# Autodesk Inventor assembly: dsitributor
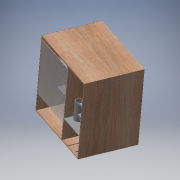
[picture p0: Inventor's stored thumbnail of the model, 180x180]
Saved by Autodesk Inventor 2019 (Build 230136000, 136)
## iProperties
Created: 2018-12-03
Part Number: dsitributor
Document SubType Name: Assembly
Designer: Bienvenue
Author: Bienvenue
## Documents named in this file (25)
- C:\Users\pouey\Desktop\rep3dM\distributeur.iam
- C:\Users\pouey\Desktop\rep3dM\planche_gauche.ipt
- C:\Users\pouey\Desktop\rep3dM\planche derrière.ipt
- C:\Users\pouey\Desktop\rep3dM\planche_bas.ipt
- C:\Users\pouey\Desktop\rep3dM\cloison_porte-monnayeur.ipt
- C:\Users\pouey\Desktop\rep3dM\monnayeur.ipt
- C:\Users\pouey\Desktop\rep3dM\cale_monnayeur.ipt
- C:\Users\pouey\Desktop\rep3dM\toboggan.ipt
- C:\Users\pouey\Desktop\rep3dM\tube.ipt
- C:\Users\pouey\Desktop\rep3dM\vis infini.ipt
- C:\Users\pouey\Desktop\rep3dM\piece-interieur-2.ipt
- C:\Users\pouey\Desktop\rep3dM\Pièce-interieur-3.ipt
- C:\Users\pouey\Desktop\rep3dM\Pièce-moteur-vis.ipt
- C:\Users\pouey\Desktop\rep3dM\vis infini_CPY.ipt
- C:\Users\pouey\Desktop\rep3dM\Pièce-moteur-vis_CPY.ipt
- C:\Users\pouey\Desktop\rep3dM\vis infini_CPY1.ipt
- C:\Users\pouey\Desktop\rep3dM\Pièce-moteur-vis_CPY1.ipt
- C:\Users\pouey\Desktop\rep3dM\vis infini_CPY2.ipt
- C:\Users\pouey\Desktop\rep3dM\Pièce-moteur-vis_CPY2.ipt
- C:\Users\pouey\Desktop\rep3dM\face-avant.ipt
- C:\Users\pouey\Desktop\rep3dM\piece-interieur4.ipt
- C:\Users\pouey\Desktop\rep3dM\vitre-avant.ipt
- C:\Users\pouey\Desktop\rep3dM\cale-moteur.ipt
- C:\Users\pouey\Desktop\rep3dM\tube-rend-monnaie.ipt
- C:\Users\pouey\Desktop\rep3dM\rampe-rendmonnaie.ipt
## Components (35 placed, 24 different names)
1. planche_gauche:1 — Mate:1, Flush:1, Flush:3, Flush:6, Mate:4, Mate:7, Placage:30, Placage:33, Placage:38, Placage:58, Placage:64, Placage:76, Placage:85
2. planche_gauche:2 — Mate:2, Flush:2, Flush:4, Flush:5, Flush:11, Placage:14, Placage:17, Placage:18, Placage:67, Placage:70, Tangente:7, Placage:90
3. planche derrière:1 — Mate:3, Flush:5, Flush:6, Mate:4, Flush:10, Placage:15, Placage:19, Placage:20, Placage:29, Placage:35, Placage:37, Placage:51, Placage:52, Placage:53, Placage:54, Placage:65, Placage:68, Placage:69, Placage:74, Placage:75, Placage:78, Placage:81, Placage:84, Tangente:6, Placage:88
4. planche_bas:1 — Mate:1, Mate:2, Flush:1, Flush:2, Flush:3, Flush:4, Mate:3, Angle:3, Placage:31, Placage:34, Placage:71, Placage:89
5. planche_bas:2 — Mate:7, Flush:10, Flush:11, Placage:16, Angle:2, Placage:21, Placage:22, Placage:57, Placage:63, Placage:77, Placage:80, Placage:87
6. cloison_porte-monnayeur:1 — Placage:14, Placage:15, Placage:16, Tangente:1, Tangente:2, Tangente:3, Tangente:4, Tangente:5, Placage:62
7. monnayeur:1 — Mate:11, Flush:14, Mate:13
8. cale_monnayeur:1 — Mate:11, Flush:14, Mate:13, Placage:17, Angle:2, Placage:19, Placage:21
9. toboggan:1 — Placage:18, Angle:3, Placage:20, Placage:22, Placage:24, Placage:25, Placage:26, Placage:27, Placage:28, Placage:66
10. tube:1 — Tangente:1, Placage:25
11. tube:2 — Placage:24, Tangente:2
12. tube:3 — Placage:26, Tangente:3
13. tube:4 — Placage:27, Tangente:4
14. tube:5 — Placage:28, Tangente:5
15. vis infini:1 — Placage:39, Placage:40, Placage:41, Angle:4, Angle:5
16. piece-interieur-2:1 — Placage:29, Placage:30, Placage:31, Placage:56, Placage:59, Placage:61, Placage:83, Placage:86
17. piece-interieur-2:2 — Placage:33, Placage:34, Placage:35, Placage:36
18. Pièce-interieur-3:1 — Placage:36, Placage:37, Placage:38, Placage:55, Placage:60, Placage:79, Placage:82
19. Pièce-moteur-vis:1 — Placage:39, Placage:40, Placage:41, Angle:4, Angle:5, Placage:51, Placage:59, Placage:60
20. vis infini_CPY:1 — Angle:6, Angle:7, Placage:42, Placage:43, Placage:44
21. Pièce-moteur-vis_CPY:1 — Angle:6, Angle:7, Placage:42, Placage:43, Placage:44, Placage:52, Placage:57, Placage:58
22. vis infini_CPY1:1 — Angle:8, Angle:9, Placage:45, Placage:46, Placage:47
23. Pièce-moteur-vis_CPY1:1 — Angle:8, Angle:9, Placage:45, Placage:46, Placage:47, Placage:53, Placage:55, Placage:56
24. vis infini_CPY2:1 — Angle:10, Angle:11, Placage:48, Placage:49, Placage:50
25. Pièce-moteur-vis_CPY2:1 — Angle:10, Angle:11, Placage:48, Placage:49, Placage:50, Placage:54, Placage:61, Placage:62
26. face-avant:1 — Placage:63, Placage:64, Placage:65, Placage:72, Placage:73
27. cale_monnayeur:2 — Placage:66, Placage:67, Placage:68
28. piece-interieur4:1 — Placage:69, Placage:70, Placage:71
29. vitre-avant:1 — Placage:72, Placage:73, Placage:74
30. cale-moteur:1 — Placage:75, Placage:76, Placage:77
31. cale-moteur:2 — Placage:78, Placage:79, Placage:80
32. cale-moteur:3 — Placage:84, Placage:85, Placage:86
33. cale-moteur:4 — Placage:81, Placage:82, Placage:83
34. tube-rend-monnaie:1 — Tangente:6, Tangente:7, Placage:87
35. rampe-rendmonnaie:1 — Placage:88, Placage:89, Placage:90
## Relationships (108: Mate 82, Angle 10, Flush 9, Tangent 7)
- Mate:1: planche_gauche:1 ↔ planche_bas:1
- Mate:2: planche_gauche:2 ↔ planche_bas:1
- Flush:1: planche_gauche:1 ↔ planche_bas:1
- Flush:2: planche_gauche:2 ↔ planche_bas:1
- Flush:3: planche_gauche:1 ↔ planche_bas:1
- Flush:4: planche_gauche:2 ↔ planche_bas:1
- Mate:3: planche derrière:1 ↔ planche_bas:1
- Flush:5: planche_gauche:2 ↔ planche derrière:1
- Flush:6: planche_gauche:1 ↔ planche derrière:1
- Mate:4: planche_gauche:1 ↔ planche derrière:1
- Mate:7: planche_gauche:1 ↔ planche_bas:2
- Flush:10: planche derrière:1 ↔ planche_bas:2
- Flush:11: planche_gauche:2 ↔ planche_bas:2
- Mate:11: monnayeur:1 ↔ cale_monnayeur:1
- Flush:14 (-50.8 mm): monnayeur:1 ↔ cale_monnayeur:1
- Mate:13: monnayeur:1 ↔ cale_monnayeur:1
- Placage:14 [Mate] (150 mm): planche_gauche:2 ↔ cloison_porte-monnayeur:1
- Placage:15 [Mate]: planche derrière:1 ↔ cloison_porte-monnayeur:1
- Placage:16 [Mate]: planche_bas:2 ↔ cloison_porte-monnayeur:1
- Placage:17 [Mate]: planche_gauche:2 ↔ cale_monnayeur:1
- Angle:2 (160 deg): planche_bas:2 ↔ cale_monnayeur:1
- Placage:18 [Mate]: planche_gauche:2 ↔ toboggan:1
- Angle:3 (180 deg): planche_bas:1 ↔ toboggan:1
- Placage:19 [Mate]: planche derrière:1 ↔ cale_monnayeur:1
- Placage:20 [Mate] (60 mm): planche derrière:1 ↔ toboggan:1
- Placage:21 [Mate] (50 mm): planche_bas:2 ↔ cale_monnayeur:1
- Placage:22 [Mate] (180 mm): planche_bas:2 ↔ toboggan:1
- Tangente:1 (10 mm): cloison_porte-monnayeur:1 ↔ tube:1
- Placage:24 [Mate]: toboggan:1 ↔ tube:2
- Tangente:2 (10 mm): cloison_porte-monnayeur:1 ↔ tube:2
- Placage:25 [Mate]: toboggan:1 ↔ tube:1
- Placage:26 [Mate]: toboggan:1 ↔ tube:3
- Tangente:3 (10 mm): cloison_porte-monnayeur:1 ↔ tube:3
- Placage:27 [Mate]: toboggan:1 ↔ tube:4
- Tangente:4 (10 mm): cloison_porte-monnayeur:1 ↔ tube:4
- Placage:28 [Mate]: toboggan:1 ↔ tube:5
- Tangente:5 (10 mm): cloison_porte-monnayeur:1 ↔ tube:5
- Placage:29 [Mate]: planche derrière:1 ↔ piece-interieur-2:1
- Placage:30 [Mate]: planche_gauche:1 ↔ piece-interieur-2:1
- Placage:31 [Mate] (250 mm): planche_bas:1 ↔ piece-interieur-2:1
- Placage:33 [Mate]: planche_gauche:1 ↔ piece-interieur-2:2
- Placage:34 [Mate] (100 mm): planche_bas:1 ↔ piece-interieur-2:2
- Placage:35 [Mate]: planche derrière:1 ↔ piece-interieur-2:2
- Placage:36 [Mate]: piece-interieur-2:2 ↔ Pièce-interieur-3:1
- Placage:37 [Mate]: planche derrière:1 ↔ Pièce-interieur-3:1
- Placage:38 [Mate] (125 mm): planche_gauche:1 ↔ Pièce-interieur-3:1
- Placage:39 [Mate]: vis infini:1 ↔ Pièce-moteur-vis:1
- Placage:40 [Mate] (-15 mm): vis infini:1 ↔ Pièce-moteur-vis:1
- Placage:41 [Mate] (5 mm): vis infini:1 ↔ Pièce-moteur-vis:1
- Angle:4 (0 deg): vis infini:1 ↔ Pièce-moteur-vis:1
- Angle:5 (90 deg): vis infini:1 ↔ Pièce-moteur-vis:1
- Angle:6 (90 deg): vis infini_CPY:1 ↔ Pièce-moteur-vis_CPY:1
- Angle:7 (0 deg): vis infini_CPY:1 ↔ Pièce-moteur-vis_CPY:1
- Placage:42 [Mate] (5 mm): vis infini_CPY:1 ↔ Pièce-moteur-vis_CPY:1
- Placage:43 [Mate] (-15 mm): vis infini_CPY:1 ↔ Pièce-moteur-vis_CPY:1
- Placage:44 [Mate]: vis infini_CPY:1 ↔ Pièce-moteur-vis_CPY:1
- Angle:8 (90 deg): vis infini_CPY1:1 ↔ Pièce-moteur-vis_CPY1:1
- Angle:9 (0 deg): vis infini_CPY1:1 ↔ Pièce-moteur-vis_CPY1:1
- Placage:45 [Mate] (5 mm): vis infini_CPY1:1 ↔ Pièce-moteur-vis_CPY1:1
- Placage:46 [Mate] (-15 mm): vis infini_CPY1:1 ↔ Pièce-moteur-vis_CPY1:1
- Placage:47 [Mate]: vis infini_CPY1:1 ↔ Pièce-moteur-vis_CPY1:1
- Angle:10 (90 deg): vis infini_CPY2:1 ↔ Pièce-moteur-vis_CPY2:1
- Angle:11 (0 deg): vis infini_CPY2:1 ↔ Pièce-moteur-vis_CPY2:1
- Placage:48 [Mate] (5 mm): vis infini_CPY2:1 ↔ Pièce-moteur-vis_CPY2:1
- Placage:49 [Mate] (-15 mm): vis infini_CPY2:1 ↔ Pièce-moteur-vis_CPY2:1
- Placage:50 [Mate]: vis infini_CPY2:1 ↔ Pièce-moteur-vis_CPY2:1
- Placage:51 [Mate] (40 mm): planche derrière:1 ↔ Pièce-moteur-vis:1
- Placage:52 [Mate] (40 mm): planche derrière:1 ↔ Pièce-moteur-vis_CPY:1
- Placage:53 [Mate] (40 mm): planche derrière:1 ↔ Pièce-moteur-vis_CPY1:1
- Placage:54 [Mate] (40 mm): planche derrière:1 ↔ Pièce-moteur-vis_CPY2:1
- Placage:55 [Mate] (20 mm): Pièce-interieur-3:1 ↔ Pièce-moteur-vis_CPY1:1
- Placage:56 [Mate] (30 mm): piece-interieur-2:1 ↔ Pièce-moteur-vis_CPY1:1
- Placage:57 [Mate] (40 mm): planche_bas:2 ↔ Pièce-moteur-vis_CPY:1
- Placage:58 [Mate] (25 mm): planche_gauche:1 ↔ Pièce-moteur-vis_CPY:1
- Placage:59 [Mate] (40 mm): piece-interieur-2:1 ↔ Pièce-moteur-vis:1
- Placage:60 [Mate] (25 mm): Pièce-interieur-3:1 ↔ Pièce-moteur-vis:1
- Placage:61 [Mate] (40 mm): piece-interieur-2:1 ↔ Pièce-moteur-vis_CPY2:1
- Placage:62 [Mate] (25 mm): cloison_porte-monnayeur:1 ↔ Pièce-moteur-vis_CPY2:1
- Placage:63 [Mate]: planche_bas:2 ↔ face-avant:1
- Placage:64 [Mate]: planche_gauche:1 ↔ face-avant:1
- Placage:65 [Mate] (300 mm): planche derrière:1 ↔ face-avant:1
- Placage:66 [Mate]: toboggan:1 ↔ cale_monnayeur:2
- Placage:67 [Mate]: planche_gauche:2 ↔ cale_monnayeur:2
- Placage:68 [Mate]: planche derrière:1 ↔ cale_monnayeur:2
- Placage:69 [Mate]: planche derrière:1 ↔ piece-interieur4:1
- Placage:70 [Mate]: planche_gauche:2 ↔ piece-interieur4:1
- Placage:71 [Mate] (115 mm): planche_bas:1 ↔ piece-interieur4:1
- Placage:72 [Mate]: face-avant:1 ↔ vitre-avant:1
- Placage:73 [Mate]: face-avant:1 ↔ vitre-avant:1
- Placage:74 [Mate] (300 mm): planche derrière:1 ↔ vitre-avant:1
- Placage:75 [Mate]: planche derrière:1 ↔ cale-moteur:1
- Placage:76 [Mate]: planche_gauche:1 ↔ cale-moteur:1
- Placage:77 [Mate]: planche_bas:2 ↔ cale-moteur:1
- Placage:78 [Mate]: planche derrière:1 ↔ cale-moteur:2
- Placage:79 [Mate]: Pièce-interieur-3:1 ↔ cale-moteur:2
- Placage:80 [Mate]: planche_bas:2 ↔ cale-moteur:2
- Placage:81 [Mate]: planche derrière:1 ↔ cale-moteur:4
- Placage:82 [Mate]: Pièce-interieur-3:1 ↔ cale-moteur:4
- Placage:83 [Mate]: piece-interieur-2:1 ↔ cale-moteur:4
- Placage:84 [Mate]: planche derrière:1 ↔ cale-moteur:3
- Placage:85 [Mate]: planche_gauche:1 ↔ cale-moteur:3
- Placage:86 [Mate]: piece-interieur-2:1 ↔ cale-moteur:3
- Tangente:6: planche derrière:1 ↔ tube-rend-monnaie:1
- Tangente:7: planche_gauche:2 ↔ tube-rend-monnaie:1
- Placage:87 [Mate] (170 mm): planche_bas:2 ↔ tube-rend-monnaie:1
- Placage:88 [Mate]: planche derrière:1 ↔ rampe-rendmonnaie:1
- Placage:89 [Mate]: planche_bas:1 ↔ rampe-rendmonnaie:1
- Placage:90 [Mate]: planche_gauche:2 ↔ rampe-rendmonnaie:1
